# Autodesk Inventor assembly: koks_v3
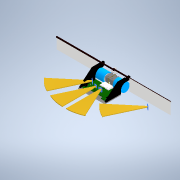
[picture p0: Inventor's stored thumbnail of the model, 180x180]
Saved by Autodesk Inventor 2022 (Build 260153000, 153)
## iProperties
Created: 2022-12-08
Part Number: koks_v3
Document SubType Name: Assembly
Designer: Kamil
Author: Kamil
## Documents named in this file (20)
- C:\MiniSumo koks\koks_v3.iam
- C:\MiniSumo koks\n20 motor.ipt
- C:\MiniSumo koks\felga.ipt
- C:\MiniSumo koks\opona.ipt
- C:\MiniSumo koks\Part8.ipt
- C:\MiniSumo koks\uchwyt na plytke.ipt
- C:\MiniSumo koks\blacha_stal_3mm.ipt
- C:\MiniSumo koks\steel_2.ipt
- C:\MiniSumo koks\lead_3.ipt
- C:\MiniSumo koks\PCB.ipt
- C:\MiniSumo koks\sciana.ipt
- C:\MiniSumo koks\strug.ipt
- C:\MiniSumo koks\sciana_MIR.ipt
- C:\MiniSumo koks\mirror.ipt
- C:\MiniSumo koks\montaz_wachlarzy.ipt
- C:\MiniSumo koks\wachlarz_1.ipt
- C:\Users\Kamil\Desktop\powerhd_hd_1370a_micro.ipt
- C:\Users\Kamil\Downloads\OLED Display 128x64.ipt
- C:\MiniSumo koks\PCB_2.ipt
- C:\MiniSumo koks\TOF_VLCOS.ipt
## Components (27 placed, 19 different names)
1. n20 motor:1 — Flush:1, Mate:1, Mate:2
2. n20 motor:2 — Flush:1, Mate:1, Mate:2, Flush:2, Flush:3, Flush:6, Flush:7
3. felga:1 — Flush:2, Flush:3
4. felga:2
5. opona:1
6. opona:2
7. Part8:1 — Flush:6, Flush:7, Flush:12, Mate:4, Angle:1, Mate:5, Flush:19, Flush:20
8. blacha_stal_3mm:1 — Flush:12, Flush:13, Mate:3, Flush:16, Flush:17, Flush:18
9. steel_2:1 — Flush:13, Flush:14, Flush:15
10. lead_3:1 — Flush:14
11. PCB:1 — Flush:15, Mate:3, Flush:16, Mate:15, Mate:16, Mate:17, Mate:18, Mate:19
12. sciana:1 — Flush:17, Flush:21
13. strug:1 — Flush:18
14. sciana_MIR:1
15. uchwyt na plytke:1 — Mate:5, Flush:19, Flush:20, Flush:22, Mate:8, Mate:9, Mate:10, Flush:24
16. mirror:1 — Flush:21
17. montaz_wachlarzy:1 — Flush:22, Flush:23, Mate:7
18. wachlarz_1:1 — Flush:23, Mate:6
19. wachlarz_1:2 — Mate:6, Mate:7
20. powerhd_hd_1370a_micro:1 — Mate:8
21. powerhd_hd_1370a_micro:2 — Mate:9
22. OLED Display 128x64:1 — Mate:10
23. PCB_2:1 — Flush:24
24. TOF_VLCOS:3 — Mate:16, Mate:17, Flush:27
25. TOF_VLCOS:4 — Mate:15, Mate:18, Flush:27, Mate:20
26. TOF_VLCOS:5 — Mate:19, Mate:20
27. TOF_VLCOS:6
## Relationships (36: Flush 19, Mate 16, Angle 1)
- Flush:1: n20 motor:1 ↔ n20 motor:2
- Mate:1 (5 mm): n20 motor:1 ↔ n20 motor:2
- Mate:2: n20 motor:1 ↔ n20 motor:2
- Flush:2: n20 motor:2 ↔ felga:1
- Flush:3: n20 motor:2 ↔ felga:1
- Flush:6: n20 motor:2 ↔ Part8:1
- Flush:7 (2.5 mm): n20 motor:2 ↔ Part8:1
- Flush:12: Part8:1 ↔ blacha_stal_3mm:1
- Flush:13: blacha_stal_3mm:1 ↔ steel_2:1
- Flush:14: steel_2:1 ↔ lead_3:1
- Flush:15 (2 mm): steel_2:1 ↔ PCB:1
- Mate:3 (0.4 mm): blacha_stal_3mm:1 ↔ PCB:1
- Flush:16 (9 mm): blacha_stal_3mm:1 ↔ PCB:1
- Flush:17: blacha_stal_3mm:1 ↔ sciana:1
- Flush:18: blacha_stal_3mm:1 ↔ strug:1
- Mate:4: Part8:1
- Angle:1 (0 deg): Part8:1
- Mate:5: Part8:1 ↔ uchwyt na plytke:1
- Flush:19: Part8:1 ↔ uchwyt na plytke:1
- Flush:20: Part8:1 ↔ uchwyt na plytke:1
- Flush:21: sciana:1 ↔ mirror:1
- Flush:22: uchwyt na plytke:1 ↔ montaz_wachlarzy:1
- Flush:23: montaz_wachlarzy:1 ↔ wachlarz_1:1
- Mate:6: wachlarz_1:1 ↔ wachlarz_1:2
- Mate:7: montaz_wachlarzy:1 ↔ wachlarz_1:2
- Mate:8: uchwyt na plytke:1 ↔ powerhd_hd_1370a_micro:1
- Mate:9: uchwyt na plytke:1 ↔ powerhd_hd_1370a_micro:2
- Mate:10 (1.5 mm): uchwyt na plytke:1 ↔ OLED Display 128x64:1
- Flush:24: uchwyt na plytke:1 ↔ PCB_2:1
- Mate:15: PCB:1 ↔ TOF_VLCOS:4
- Mate:16: PCB:1 ↔ TOF_VLCOS:3
- Mate:17: PCB:1 ↔ TOF_VLCOS:3
- Mate:18: PCB:1 ↔ TOF_VLCOS:4
- Flush:27: TOF_VLCOS:3 ↔ TOF_VLCOS:4
- Mate:19: PCB:1 ↔ TOF_VLCOS:5
- Mate:20 (23 mm): TOF_VLCOS:4 ↔ TOF_VLCOS:5
